# Autodesk Inventor assembly: GFRP_T2_11
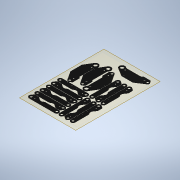
[picture p0: Inventor's stored thumbnail of the model, 180x180]
Saved by Autodesk Inventor 2020 (Build 240168000, 168)
## iProperties
Created: 2021-08-27
Part Number: GFRP_T2_11
Document SubType Name: Assembly
Designer: Masato
Author: Masato
## Documents named in this file (4)
- D:\GitHub\inventor\SUSTAINA-OP\Cam\GFRP_T2_11.iam
- D:\GitHub\inventor\SUSTAINA-OP\Cam\DisposableBoard.ipt
- D:\GitHub\inventor\SUSTAINA-OP\LowerBody\Link\BackLink_frame.ipt
- D:\GitHub\inventor\SUSTAINA-OP\LowerBody\Link\FrontLink_frame.ipt
## Components (17 placed, 3 different names)
1. DisposableBoard:1 — メイト:2, メイト:1, フラッシュ:1, フラッシュ:2, メイト:4, メイト:5, フラッシュ:3, 正接:1, 正接:2, 角度:1, メイト:7, 正接:3, メイト:8, 正接:5, メイト:11, メイト:12, メイト:14, メイト:16, メイト:19, メイト:21, 正接:9
2. FrontLink_frame:1 — メイト:11, メイト:18, 正接:6
3. FrontLink_frame:2 — メイト:12, メイト:19, 正接:7, メイト:20, 正接:8
4. FrontLink_frame:3 — メイト:14, メイト:20, 正接:8
5. FrontLink_frame:4 — メイト:16, メイト:21, 正接:9
6. BackLink_frame:1 — メイト:4, メイト:6, 正接:2
7. BackLink_frame:2 — メイト:5, フラッシュ:3, メイト:6, 正接:1, 正接:4
8. BackLink_frame:4
9. BackLink_frame:5
10. BackLink_frame:6 — 正接:6, 正接:7
11. BackLink_frame:7
12. BackLink_frame:9 — メイト:8, メイト:9, 正接:5
13. BackLink_frame:11
14. BackLink_frame:8 — 角度:1, メイト:7, 正接:3, 正接:4, メイト:9
15. BackLink_frame:10
16. BackLink_frame:12 — メイト:18
17. BackLink_frame:13
## Component patterns: (3 elements, first: BackLink_frame:1 + BackLink_frame:2), (2 elements, first: BackLink_frame:9), (2 elements, first: BackLink_frame:8), コンポーネント パターン 5:2 (2 elements)
## Relationships (29: Mate 16, Tangent 9, Flush 3, Angle 1)
- メイト:2 [Mate]: DisposableBoard:1
- メイト:1 [Mate]: DisposableBoard:1
- フラッシュ:1 [Flush]: DisposableBoard:1
- フラッシュ:2 [Flush]: DisposableBoard:1
- メイト:4 [Mate]: DisposableBoard:1 ↔ BackLink_frame:1
- メイト:5 [Mate]: DisposableBoard:1 ↔ BackLink_frame:2
- フラッシュ:3 [Flush] (2 mm): DisposableBoard:1 ↔ BackLink_frame:2
- メイト:6 [Mate] (2.5 mm): BackLink_frame:1 ↔ BackLink_frame:2
- 正接:1 [Tangent] (2 mm): DisposableBoard:1 ↔ BackLink_frame:2
- 正接:2 [Tangent] (2 mm): DisposableBoard:1 ↔ BackLink_frame:1
- 角度:1 [Angle] (0 deg): DisposableBoard:1 ↔ BackLink_frame:8
- メイト:7 [Mate]: DisposableBoard:1 ↔ BackLink_frame:8
- 正接:3 [Tangent] (2 mm): DisposableBoard:1 ↔ BackLink_frame:8
- 正接:4 [Tangent] (2.5 mm): BackLink_frame:2 ↔ BackLink_frame:8
- メイト:8 [Mate]: DisposableBoard:1 ↔ BackLink_frame:9
- メイト:9 [Mate] (2.5 mm): BackLink_frame:9 ↔ BackLink_frame:8
- 正接:5 [Tangent] (2 mm): DisposableBoard:1 ↔ BackLink_frame:9
- メイト:11 [Mate]: DisposableBoard:1 ↔ FrontLink_frame:1
- メイト:12 [Mate]: DisposableBoard:1 ↔ FrontLink_frame:2
- メイト:14 [Mate]: DisposableBoard:1 ↔ FrontLink_frame:3
- メイト:16 [Mate]: DisposableBoard:1 ↔ FrontLink_frame:4
- メイト:18 [Mate] (2.5 mm): FrontLink_frame:1 ↔ BackLink_frame:12
- 正接:6 [Tangent] (2.5 mm): FrontLink_frame:1 ↔ BackLink_frame:6
- メイト:19 [Mate] (2 mm): DisposableBoard:1 ↔ FrontLink_frame:2
- 正接:7 [Tangent] (2.5 mm): FrontLink_frame:2 ↔ BackLink_frame:6
- メイト:20 [Mate] (2.5 mm): FrontLink_frame:2 ↔ FrontLink_frame:3
- 正接:8 [Tangent] (2.5 mm): FrontLink_frame:2 ↔ FrontLink_frame:3
- メイト:21 [Mate] (2.5 mm): DisposableBoard:1 ↔ FrontLink_frame:4
- 正接:9 [Tangent] (3 mm): DisposableBoard:1 ↔ FrontLink_frame:4
